# Autodesk Inventor assembly: SAR330 + coupler right bracket
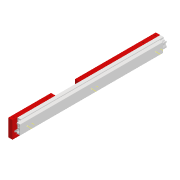
[picture p0: Inventor's stored thumbnail of the model, 180x180]
Saved by Autodesk Inventor 2020 (Build 240168000, 168)
## iProperties
Created: 2019-12-26
Part Number: SAR330 + coupler right bracket
Document SubType Name: Assembly
Designer: ball
Author: ball
## Documents named in this file (4)
- C:\FTC\FTC8863CAD\2019 Robot\Delivery\Lift Right\SAR330 + coupler right bracket.iam
- C:\FTC\FTC8863CAD\Misumi\SAR330\SAR330 440 offset.iam
- C:\FTC\FTC8863CAD\2019 Robot\Delivery\Lift Right\Coupler lift short right + pulleys.iam
- C:\FTC\FTC8863CAD\2019 Robot\Delivery\Lift Right\Coupler lift long right bracket + pulley.iam
## Components (3 placed, 3 different names)
1. SAR330 440 offset:1 [sub-assembly] — Mate:1, Mate:2, Flush:1, Mate:3, Mate:4, Mate:5
2. Coupler lift short right + pulleys:1 [sub-assembly] — Mate:1, Mate:2, Flush:1
3. Coupler lift long right bracket + pulley:2 [sub-assembly] — Mate:3, Mate:4, Mate:5
## Relationships (6: Mate 5, Flush 1)
- Mate:1: SAR330 440 offset:1 ↔ Coupler lift short right + pulleys:1
- Mate:2: SAR330 440 offset:1 ↔ Coupler lift short right + pulleys:1
- Flush:1: SAR330 440 offset:1 ↔ Coupler lift short right + pulleys:1
- Mate:3: SAR330 440 offset:1 ↔ Coupler lift long right bracket + pulley:2
- Mate:4: SAR330 440 offset:1 ↔ Coupler lift long right bracket + pulley:2
- Mate:5: SAR330 440 offset:1 ↔ Coupler lift long right bracket + pulley:2
